# Autodesk Inventor assembly: DoubleSlipHR_printasm
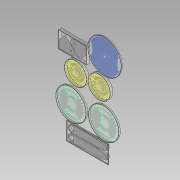
[picture p0: Inventor's stored thumbnail of the model, 180x180]
Saved by Autodesk Inventor 2021 (Build 250183000, 183)
## iProperties
Created: 2021-05-13
Part Number: DoubleSlipHR_printasm
Document SubType Name: Assembly
Designer: kumagai
Author: kumagai
## Documents named in this file (7)
- X:\Develop\CAD\PlaRails\DoubleSlip\DoubleSlipHR_printasm.iam
- X:\Develop\CAD\PlaRails\DoubleSlip\DoubleSlipHR_printbase.ipt
- X:\Develop\CAD\PlaRails\DoubleSlip\GearBarBase.ipt
- X:\Develop\CAD\PlaRails\DoubleSlip\GearCenter.ipt
- X:\Develop\CAD\PlaRails\DoubleSlip\GearCenterCover.ipt
- X:\Develop\CAD\PlaRails\DoubleSlip\DSHR_BarCover.ipt
- X:\Develop\CAD\PlaRails\DoubleSlip\DoubleSlipHR_Bar.ipt
## Components (10 placed, 6 different names)
1. DoubleSlipHR_printbase:1 — メイト:3, メイト:4, メイト:7, メイト:8, メイト:10, メイト:13, メイト:14, メイト:15, メイト:16, メイト:18, メイト:19
2. GearBarBase:1 — メイト:5, メイト:8
3. GearBarBase:2 — メイト:6, メイト:7
4. GearCenter:1 — メイト:1, メイト:3
5. GearCenter:2 — メイト:2, メイト:4
6. GearCenterCover:1 — メイト:9, メイト:10
7. DSHR_BarCover:1 — メイト:12, メイト:13, メイト:14
8. DSHR_BarCover:2 — メイト:11, メイト:15, メイト:16
9. DoubleSlipHR_Bar:2 — メイト:17, メイト:18, メイト:19
10. DoubleSlipHR_Bar:3
## Component patterns: (2 elements, first: DoubleSlipHR_Bar:2)
## Relationships (19: Mate 19)
- メイト:1 [Mate]: GearCenter:1
- メイト:2 [Mate]: GearCenter:2
- メイト:3 [Mate]: DoubleSlipHR_printbase:1 ↔ GearCenter:1
- メイト:4 [Mate]: DoubleSlipHR_printbase:1 ↔ GearCenter:2
- メイト:5 [Mate]: GearBarBase:1
- メイト:6 [Mate]: GearBarBase:2
- メイト:7 [Mate]: DoubleSlipHR_printbase:1 ↔ GearBarBase:2
- メイト:8 [Mate]: DoubleSlipHR_printbase:1 ↔ GearBarBase:1
- メイト:9 [Mate]: GearCenterCover:1
- メイト:10 [Mate]: DoubleSlipHR_printbase:1 ↔ GearCenterCover:1
- メイト:11 [Mate]: DSHR_BarCover:2
- メイト:12 [Mate]: DSHR_BarCover:1
- メイト:13 [Mate] (0.8 mm): DoubleSlipHR_printbase:1 ↔ DSHR_BarCover:1
- メイト:14 [Mate] (0.8 mm): DoubleSlipHR_printbase:1 ↔ DSHR_BarCover:1
- メイト:15 [Mate] (0.8 mm): DoubleSlipHR_printbase:1 ↔ DSHR_BarCover:2
- メイト:16 [Mate] (0.8 mm): DoubleSlipHR_printbase:1 ↔ DSHR_BarCover:2
- メイト:17 [Mate]: DoubleSlipHR_Bar:2
- メイト:18 [Mate] (0.8 mm): DoubleSlipHR_printbase:1 ↔ DoubleSlipHR_Bar:2
- メイト:19 [Mate] (5.3 mm): DoubleSlipHR_printbase:1 ↔ DoubleSlipHR_Bar:2
